# Autodesk Inventor assembly: Pergola top gouble spaced
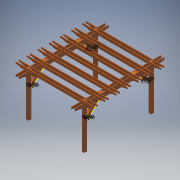
[picture p0: Inventor's stored thumbnail of the model, 180x180]
Saved by Autodesk Inventor 2016 (Build 200138000, 138)
## iProperties
Created: 2014-06-08
Part Number: Pergola top gouble spaced
Document SubType Name: Assembly
Designer: Haden
Author: Haden
## Documents named in this file (8)
- C:\Users\Haden\Desktop\Desktop\CAD\Pergola\Pergola top double spaced.iam
- C:\Users\Haden\Desktop\Desktop\CAD\Pergola\Post.ipt
- C:\Users\Haden\Desktop\Desktop\CAD\Pergola\Support Beam.ipt
- C:\Users\Haden\Desktop\Desktop\CAD\Pergola\Cover Board.ipt
- C:\Users\Haden\Desktop\Desktop\CAD\Pergola\Top Board.ipt
- C:\Users\Haden\Desktop\Desktop\CAD\Pergola\Angled Support.ipt
- C:\Users\Haden\Desktop\Desktop\CAD\Pergola\Angled Support Attachment.ipt
- C:\Users\Haden\Desktop\Desktop\CAD\Pergola\Angle Brace Knob.ipt
## Components (46 placed, 7 different names)
1. Post:1 — Flush:1, Flush:2, Flush:3, Flush:4, Flush:5, Flush:8, Flush:9, Mate:10, Mate:11, Flush:52, Mate:28
2. Post:2 — Flush:1, Flush:5, Flush:6, Flush:9, Mate:29
3. Post:3 — Flush:2, Flush:6, Flush:7, Mate:19, Mate:27
4. Post:4 — Flush:3, Flush:4, Flush:7, Flush:8, Mate:8, Mate:9, Flush:33, Mate:12, Mate:13, Flush:40, Flush:41, Mate:17, Flush:43, Flush:51, Mate:18, Mate:23
5. Support Beam:1 — Flush:27, Flush:30, Mate:8, Flush:33, Mate:16, Flush:53
6. Support Beam:2 — Flush:27, Flush:28, Flush:30, Flush:31, Mate:9
7. Support Beam:3 — Flush:28, Flush:29, Flush:31, Flush:32, Mate:10
8. Support Beam:4 — Flush:29, Flush:32, Mate:11
9. Angled Support:1 — Flush:44, Flush:46, Flush:48, Flush:49, Flush:51, Mate:18, Flush:53, Flush:55, Mate:22, Mate:33
10. Angled Support:2 — Flush:44, Flush:46, Flush:50, Flush:52, Flush:56, Mate:24, Mate:30
11. Angled Support:3 — Flush:45, Flush:47, Flush:48, Flush:49, Mate:19, Flush:58, Mate:25, Mate:32
12. Angled Support:4 — Flush:45, Flush:47, Flush:50, Flush:57, Mate:26, Mate:31
13. Angled Support Attachment:1 — Flush:55, Mate:22, Mate:23, Flush:59, Flush:60
14. Angled Support Attachment:2 — Flush:58, Mate:25, Mate:27, Flush:65, Flush:66
15. Angled Support Attachment:3 — Flush:57, Mate:26, Mate:29, Flush:63, Flush:64
16. Angled Support Attachment:4 — Flush:56, Mate:24, Mate:28, Flush:61, Flush:62
17. Angle Brace Knob:1 — Mate:30, Flush:61, Flush:62
18. Angle Brace Knob:2 — Mate:31, Flush:63, Flush:64
19. Angle Brace Knob:3 — Mate:32, Flush:65, Flush:66
20. Angle Brace Knob:4 — Mate:33, Flush:59, Flush:60
21. Cover Board:1 — Flush:34, Flush:37, Mate:12, Flush:40, Flush:41, Mate:16, Flush:42
22. Cover Board:2 — Flush:34, Flush:37, Mate:13
23. Cover Board:5
24. Cover Board:6
25. Cover Board:7
26. Cover Board:8
27. Cover Board:9
28. Cover Board:10
29. Cover Board:11
30. Cover Board:12
31. Cover Board:13
32. Cover Board:14
33. Cover Board:15
34. Cover Board:16 — Mate:20
35. Top Board:2 — Mate:20, Flush:54, Mate:21
36. Top Board:1 — Mate:17, Flush:42, Flush:43, Flush:54, Mate:21
37. Top Board:3
38. Top Board:4
39. Top Board:5
40. Top Board:6
41. Top Board:7
42. Top Board:8
43. Top Board:9
44. Top Board:10
45. Top Board:11
46. Top Board:12
## Component patterns: (7 elements, first: Cover Board:1 + Cover Board:2), (6 elements, first: Top Board:2 + Top Board:1)
## Relationships (69: Flush 45, Mate 24)
- Flush:1: Post:1 ↔ Post:2
- Flush:2: Post:1 ↔ Post:3
- Flush:3: Post:1 ↔ Post:4
- Flush:4: Post:1 ↔ Post:4
- Flush:5: Post:1 ↔ Post:2
- Flush:6: Post:2 ↔ Post:3
- Flush:7: Post:3 ↔ Post:4
- Flush:8 (3048 mm): Post:1 ↔ Post:4
- Flush:9 (3657.6 mm): Post:1 ↔ Post:2
- Flush:27: Support Beam:1 ↔ Support Beam:2
- Flush:28: Support Beam:2 ↔ Support Beam:3
- Flush:29: Support Beam:3 ↔ Support Beam:4
- Flush:30: Support Beam:1 ↔ Support Beam:2
- Flush:31: Support Beam:2 ↔ Support Beam:3
- Flush:32: Support Beam:3 ↔ Support Beam:4
- Mate:8: Post:4 ↔ Support Beam:1
- Mate:9: Post:4 ↔ Support Beam:2
- Mate:10: Post:1 ↔ Support Beam:3
- Mate:11: Post:1 ↔ Support Beam:4
- Flush:33 (-539.75 mm): Post:4 ↔ Support Beam:1
- Flush:34: Cover Board:1 ↔ Cover Board:2
- Flush:37: Cover Board:1 ↔ Cover Board:2
- Mate:12: Post:4 ↔ Cover Board:1
- Mate:13: Post:4 ↔ Cover Board:2
- Flush:40 (-25.4 mm): Post:4 ↔ Cover Board:1
- Flush:41: Post:4 ↔ Cover Board:1
- Mate:16: Support Beam:1 ↔ Cover Board:1
- Mate:17: Post:4 ↔ Top Board:1
- Flush:42: Cover Board:1 ↔ Top Board:1
- Flush:43: Post:4 ↔ Top Board:1
- Flush:44: Angled Support:1 ↔ Angled Support:2
- Flush:45: Angled Support:3 ↔ Angled Support:4
- Flush:46: Angled Support:1 ↔ Angled Support:2
- Flush:47: Angled Support:3 ↔ Angled Support:4
- Flush:48: Angled Support:1 ↔ Angled Support:3
- Flush:49: Angled Support:1 ↔ Angled Support:3
- Flush:50: Angled Support:2 ↔ Angled Support:4
- Flush:51: Post:4 ↔ Angled Support:1
- Flush:52: Post:1 ↔ Angled Support:2
- Mate:18: Post:4 ↔ Angled Support:1
- Mate:19: Post:3 ↔ Angled Support:3
- Flush:53: Support Beam:1 ↔ Angled Support:1
- Mate:20: Cover Board:16 ↔ Top Board:2
- Flush:54: Top Board:2 ↔ Top Board:1
- Mate:21 (114.3 mm): Top Board:2 ↔ Top Board:1
- Flush:55 (25.4 mm): Angled Support:1 ↔ Angled Support Attachment:1
- Mate:22: Angled Support:1 ↔ Angled Support Attachment:1
- Mate:23: Post:4 ↔ Angled Support Attachment:1
- Flush:56: Angled Support:2 ↔ Angled Support Attachment:4
- Flush:57 (25.4 mm): Angled Support:4 ↔ Angled Support Attachment:3
- Flush:58 (25.4 mm): Angled Support:3 ↔ Angled Support Attachment:2
- Mate:24: Angled Support:2 ↔ Angled Support Attachment:4
- Mate:25: Angled Support:3 ↔ Angled Support Attachment:2
- Mate:26: Angled Support:4 ↔ Angled Support Attachment:3
- Mate:27: Post:3 ↔ Angled Support Attachment:2
- Mate:28: Post:1 ↔ Angled Support Attachment:4
- Mate:29: Post:2 ↔ Angled Support Attachment:3
- Mate:30: Angled Support:2 ↔ Angle Brace Knob:1
- Mate:31: Angled Support:4 ↔ Angle Brace Knob:2
- Mate:32: Angled Support:3 ↔ Angle Brace Knob:3
- Mate:33: Angled Support:1 ↔ Angle Brace Knob:4
- Flush:59: Angled Support Attachment:1 ↔ Angle Brace Knob:4
- Flush:60: Angled Support Attachment:1 ↔ Angle Brace Knob:4
- Flush:61: Angled Support Attachment:4 ↔ Angle Brace Knob:1
- Flush:62: Angled Support Attachment:4 ↔ Angle Brace Knob:1
- Flush:63: Angled Support Attachment:3 ↔ Angle Brace Knob:2
- Flush:64: Angled Support Attachment:3 ↔ Angle Brace Knob:2
- Flush:65: Angled Support Attachment:2 ↔ Angle Brace Knob:3
- Flush:66: Angled Support Attachment:2 ↔ Angle Brace Knob:3
